# Autodesk Inventor assembly: Default Motor Testbench Mk2
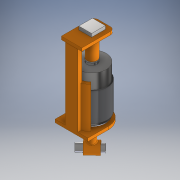
[picture p0: Inventor's stored thumbnail of the model, 180x180]
Saved by Autodesk Inventor 2018 (Build 220112000, 112)
## iProperties
Created: 2018-01-11
Part Number: Default Motor Testbench Mk2
Document SubType Name: Assembly
Designer: Moochster
Author: Moochster
## Documents named in this file (8)
- C:\Users\Moochster\OneDrive\Documents\2018 UBC\ELEC 391\Controller\CAD\Default Motor Testbench Mk2.iam
- C:\Users\Moochster\OneDrive\Documents\2018 UBC\ELEC 391\Controller\CAD\JD5B-2655W-R.ipt
- C:\Users\Moochster\OneDrive\Documents\2018 UBC\ELEC 391\Controller\CAD\Motor Face Mount.ipt
- C:\Users\Moochster\OneDrive\Documents\2018 UBC\ELEC 391\Controller\CAD\Laser Mount.ipt
- C:\Users\Moochster\OneDrive\Documents\2018 UBC\ELEC 391\Controller\CAD\Motor Rotary Encoder Coupler.ipt
- C:\Users\Moochster\OneDrive\Documents\2018 UBC\ELEC 391\Controller\CAD\VLM-650-03-LPT.ipt
- C:\Users\Moochster\OneDrive\Documents\2018 UBC\ELEC 391\Controller\CAD\PEC12R-4017F-N0024.iam
- C:\Users\Moochster\OneDrive\Documents\2018 UBC\ELEC 391\Controller\CAD\Rotary Encoder Mount.ipt
## Components (7 placed, 7 different names)
1. JD5B-2655W-R:1 — Mate:1, Mate:4, Mate:5, Mate:7
2. Motor Face Mount:1 — Mate:1, Mate:2, Mate:4, Angle:3, Flush:1
3. Laser Mount:1 — Mate:5, Mate:6
4. Motor Rotary Encoder Coupler:1 — Mate:7, Mate:8, Angle:1, Angle:2
5. VLM-650-03-LPT:1 — Mate:6
6. PEC12R-4017F-N0024:1 [sub-assembly] — Mate:8, Angle:1, Angle:2, Angle:3, Mate:9
7. Rotary Encoder Mount:1 — Mate:9, Flush:1
## Relationships (12: Mate 8, Angle 3, Flush 1)
- Mate:1: JD5B-2655W-R:1 ↔ Motor Face Mount:1
- Mate:2: Motor Face Mount:1
- Mate:4: JD5B-2655W-R:1 ↔ Motor Face Mount:1
- Mate:5: JD5B-2655W-R:1 ↔ Laser Mount:1
- Mate:6: Laser Mount:1 ↔ VLM-650-03-LPT:1
- Mate:7: JD5B-2655W-R:1 ↔ Motor Rotary Encoder Coupler:1
- Mate:8: Motor Rotary Encoder Coupler:1 ↔ PEC12R-4017F-N0024:1
- Angle:1 (0 deg): Motor Rotary Encoder Coupler:1 ↔ PEC12R-4017F-N0024:1
- Angle:2 (180 deg): Motor Rotary Encoder Coupler:1 ↔ PEC12R-4017F-N0024:1
- Angle:3 (0 deg): Motor Face Mount:1 ↔ PEC12R-4017F-N0024:1
- Mate:9: PEC12R-4017F-N0024:1 ↔ Rotary Encoder Mount:1
- Flush:1: Motor Face Mount:1 ↔ Rotary Encoder Mount:1
